# Autodesk Inventor assembly: ModularGripper
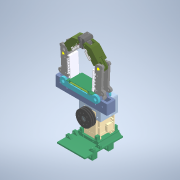
[picture p0: Inventor's stored thumbnail of the model, 180x180]
Saved by Autodesk Inventor 2020 (Build 240168000, 168)
## iProperties
Created: 2020-05-08
Part Number: ModularGripper
Document SubType Name: Assembly
Designer: Ajay Yadiki
Author: Ajay Yadiki
## Documents named in this file (10)
- C:\Users\Ajay Yadiki\Desktop\Project Gripper\ModularGripper.iam
- C:\Users\Ajay Yadiki\Desktop\Project Gripper\Motor_Base.ipt
- C:\Users\Ajay Yadiki\Desktop\Project Gripper\MotorMX-64AT_AR.ipt
- C:\Users\Ajay Yadiki\Desktop\Project Gripper\MotorCasing.ipt
- C:\Users\Ajay Yadiki\Desktop\Project Gripper\GripperBase.ipt
- C:\Users\Ajay Yadiki\Desktop\Project Gripper\MainPhalangeAssembly.iam
- C:\Users\Ajay Yadiki\Desktop\Project Gripper\EndPhalangeAssembly.iam
- C:\Users\Ajay Yadiki\Desktop\Project Gripper\Nail.ipt
- C:\Users\Ajay Yadiki\Desktop\Project Gripper\PulleyAssembly.iam
- C:\Users\Ajay Yadiki\Desktop\Project Gripper\Palm.iam
## Components (12 placed, 9 different names)
1. Motor_Base:1 — Mate:1, Mate:2, Mate:3
2. MotorMX-64AT_AR:1 — Mate:1, Mate:2, Mate:3, Mate:4, Mate:5, Mate:6, Mate:22, Mate:23, Mate:24
3. MotorCasing:1 — Mate:4, Mate:5, Mate:6, Mate:7, Mate:8, Mate:9
4. GripperBase:1 — Mate:7, Mate:8, Mate:9, Mate:10, Mate:11, Mate:12, Mate:13, Mate:25, Mate:26, Mate:27
5. MainPhalangeAssembly:1 [sub-assembly] — Mate:12, Mate:13, Mate:30, Mate:31
6. MainPhalangeAssembly:2 [sub-assembly] — Mate:10, Mate:11, Mate:28, Mate:29
7. EndPhalangeAssembly:1 [sub-assembly] — Mate:30, Mate:31, Mate:32, Mate:35
8. EndPhalangeAssembly:2 [sub-assembly] — Mate:28, Mate:29, Mate:33, Mate:34
9. Nail:1 — Mate:32, Mate:35
10. Nail:2 — Mate:33, Mate:34
11. PulleyAssembly:1 [sub-assembly] — Mate:22, Mate:23, Mate:24
12. Palm:1 [sub-assembly] — Mate:25, Mate:26, Mate:27
## Relationships (27: Mate 27)
- Mate:1: Motor_Base:1 ↔ MotorMX-64AT_AR:1
- Mate:2: Motor_Base:1 ↔ MotorMX-64AT_AR:1
- Mate:3: Motor_Base:1 ↔ MotorMX-64AT_AR:1
- Mate:4: MotorMX-64AT_AR:1 ↔ MotorCasing:1
- Mate:5: MotorMX-64AT_AR:1 ↔ MotorCasing:1
- Mate:6: MotorMX-64AT_AR:1 ↔ MotorCasing:1
- Mate:7: MotorCasing:1 ↔ GripperBase:1
- Mate:8: MotorCasing:1 ↔ GripperBase:1
- Mate:9: MotorCasing:1 ↔ GripperBase:1
- Mate:10: GripperBase:1 ↔ MainPhalangeAssembly:2
- Mate:11 (0.5 mm): GripperBase:1 ↔ MainPhalangeAssembly:2
- Mate:12: GripperBase:1 ↔ MainPhalangeAssembly:1
- Mate:13 (0.5 mm): GripperBase:1 ↔ MainPhalangeAssembly:1
- Mate:22: MotorMX-64AT_AR:1 ↔ PulleyAssembly:1
- Mate:23: MotorMX-64AT_AR:1 ↔ PulleyAssembly:1
- Mate:24: MotorMX-64AT_AR:1 ↔ PulleyAssembly:1
- Mate:25: GripperBase:1 ↔ Palm:1
- Mate:26: GripperBase:1 ↔ Palm:1
- Mate:27 (0.3 mm): GripperBase:1 ↔ Palm:1
- Mate:28: MainPhalangeAssembly:2 ↔ EndPhalangeAssembly:2
- Mate:29 (0.5 mm): MainPhalangeAssembly:2 ↔ EndPhalangeAssembly:2
- Mate:30: MainPhalangeAssembly:1 ↔ EndPhalangeAssembly:1
- Mate:31 (0.5 mm): MainPhalangeAssembly:1 ↔ EndPhalangeAssembly:1
- Mate:32: EndPhalangeAssembly:1 ↔ Nail:1
- Mate:33: EndPhalangeAssembly:2 ↔ Nail:2
- Mate:34 (0.5 mm): EndPhalangeAssembly:2 ↔ Nail:2
- Mate:35 (0.5 mm): EndPhalangeAssembly:1 ↔ Nail:1
